# Autodesk Inventor assembly: motormountsupportv1jig
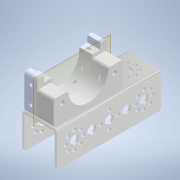
[picture p0: Inventor's stored thumbnail of the model, 180x180]
Saved by Autodesk Inventor 2020.1 (Build 241239000, 239)
## iProperties
Created: 2019-11-25
Part Number: motormountsupportv1jig
Document SubType Name: Assembly
Designer: tbloo
Author: tbloo
## Documents named in this file (4)
- C:\Users\tbloo\Documents\GitHub\AO_Robotics\CAD\Projects\Timothy Bloot\motormountsupportv1jig.iam
- C:\Users\tbloo\Documents\GitHub\AO_Robotics\CAD\Parts Kits\FTC Tetrix KOP Organized (7-24-19)\Frame Hardware\Tetrix_39066.ipt
- C:\Users\tbloo\Documents\GitHub\AO_Robotics\CAD\Parts Kits\FTC Tetrix KOP Organized (7-24-19)\Motor\739376\Tetrix_739376_Base.ipt
- C:\Users\tbloo\Documents\Part1.ipt
## Components (3 placed, 3 different names)
1. Tetrix_39066:1 — Rigid:1
2. Tetrix_739376_Base:1 — Rigid:1, Flush:1
3. Part1:1 — Flush:1
## Relationships (2: WeldJoint 1, Flush 1)
- Rigid:1 [WeldJoint]: Tetrix_39066:1 ↔ Tetrix_739376_Base:1
- Flush:1: Tetrix_739376_Base:1 ↔ Part1:1
